# Autodesk Inventor assembly: case v3
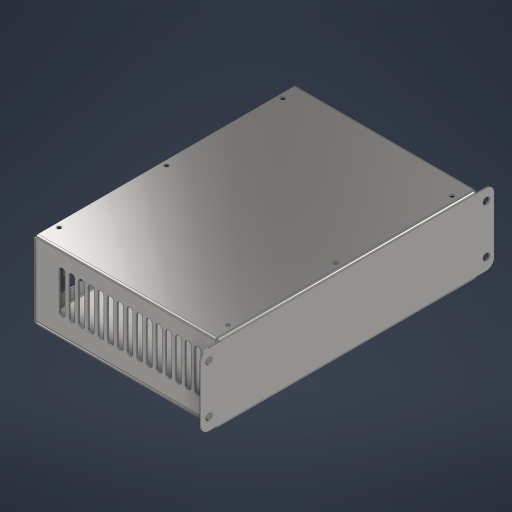
[picture p0: Inventor's stored thumbnail of the model, 512x512]
Saved by Autodesk Inventor 2024.2 (Build 282272000, 272)
## iProperties
Created: 2025-01-23
Part Number: case v3
Document SubType Name: Assembly
Designer: voids
Author: voids
## Documents named in this file (7)
- C:\Users\voids\Documents\GitHub\drive-hardware-dev\manufacturing\case v3.iam
- C:\Users\voids\Documents\GitHub\drive-hardware-dev\manufacturing\case v3 cover.ipt
- C:\Users\voids\Documents\GitHub\drive-hardware-dev\manufacturing\case v3.ipt
- C:\Users\voids\Documents\GitHub\drive-hardware-dev\manufacturing\simple step\HV servo drive v1r2\HV servo drive v1_PCB.ipt
- C:\Users\voids\Documents\GitHub\drive-hardware-dev\manufacturing\SanAce_9GA_40x20_RBD.ipt
- C:\Users\voids\Documents\GitHub\drive-hardware-dev\manufacturing\simple step\95185A110_Zinc-Plated Steel Press-Fit Nut for Sheet Metal\95185A110_Zinc-Plated Steel Press-Fit Nut for Sheet Metal.ipt
- C:\Users\voids\Documents\GitHub\drive-hardware-dev\manufacturing\simple step\95185A340_Zinc-Plated Steel Press-Fit Nut for Sheet Metal\95185A340_Zinc-Plated Steel Press-Fit Nut for Sheet Metal.ipt
## Components (16 placed, 6 different names)
1. case v3 cover:1 — Rigid:3, Rigid:10, Rigid:11, Rigid:12, Rigid:13
2. case v3:1 — Mate:1, Mate:2, Flush:1, Rigid:1, Rigid:2, Rigid:3, Rigid:4, Rigid:5, Rigid:6, Rigid:7, Rigid:8, Rigid:9, Rotational:1
3. HV servo drive v1_PCB:1 — Mate:1, Mate:2, Flush:1
4. SanAce_9GA_40x20_RBD:1 — Rigid:1
5. SanAce_9GA_40x20_RBD:2 — Rigid:2
6. 95185A110_Zinc-Plated Steel Press-Fit Nut for Sheet Metal:1 — Rigid:5
7. 95185A110_Zinc-Plated Steel Press-Fit Nut for Sheet Metal:2 — Rigid:7
8. 95185A110_Zinc-Plated Steel Press-Fit Nut for Sheet Metal:3 — Rigid:6
9. 95185A110_Zinc-Plated Steel Press-Fit Nut for Sheet Metal:4 — Rigid:8
10. 95185A110_Zinc-Plated Steel Press-Fit Nut for Sheet Metal:5 — Rigid:9
11. 95185A110_Zinc-Plated Steel Press-Fit Nut for Sheet Metal:6 — Rigid:10
12. 95185A110_Zinc-Plated Steel Press-Fit Nut for Sheet Metal:7 — Rigid:12
13. 95185A110_Zinc-Plated Steel Press-Fit Nut for Sheet Metal:8 — Rigid:13
14. 95185A110_Zinc-Plated Steel Press-Fit Nut for Sheet Metal:9 — Rigid:11
15. 95185A110_Zinc-Plated Steel Press-Fit Nut for Sheet Metal:10 — Rigid:4
16. 95185A340_Zinc-Plated Steel Press-Fit Nut for Sheet Metal:1 — Rotational:1
## Relationships (17: WeldJoint 13, Mate 2, Flush 1, RevoluteJoint 1)
- Mate:1 (7.9375 mm): case v3:1 ↔ HV servo drive v1_PCB:1
- Mate:2: case v3:1 ↔ HV servo drive v1_PCB:1
- Flush:1: case v3:1 ↔ HV servo drive v1_PCB:1
- Rigid:1 [WeldJoint]: case v3:1 ↔ SanAce_9GA_40x20_RBD:1
- Rigid:2 [WeldJoint]: case v3:1 ↔ SanAce_9GA_40x20_RBD:2
- Rigid:3 [WeldJoint]: case v3 cover:1 ↔ case v3:1
- Rigid:4 [WeldJoint]: case v3:1 ↔ 95185A110_Zinc-Plated Steel Press-Fit Nut for Sheet Metal:10
- Rigid:5 [WeldJoint]: case v3:1 ↔ 95185A110_Zinc-Plated Steel Press-Fit Nut for Sheet Metal:1
- Rigid:6 [WeldJoint]: case v3:1 ↔ 95185A110_Zinc-Plated Steel Press-Fit Nut for Sheet Metal:3
- Rigid:7 [WeldJoint]: case v3:1 ↔ 95185A110_Zinc-Plated Steel Press-Fit Nut for Sheet Metal:2
- Rigid:8 [WeldJoint]: case v3:1 ↔ 95185A110_Zinc-Plated Steel Press-Fit Nut for Sheet Metal:4
- Rigid:9 [WeldJoint]: case v3:1 ↔ 95185A110_Zinc-Plated Steel Press-Fit Nut for Sheet Metal:5
- Rigid:10 [WeldJoint]: case v3 cover:1 ↔ 95185A110_Zinc-Plated Steel Press-Fit Nut for Sheet Metal:6
- Rigid:11 [WeldJoint]: case v3 cover:1 ↔ 95185A110_Zinc-Plated Steel Press-Fit Nut for Sheet Metal:9
- Rigid:12 [WeldJoint]: case v3 cover:1 ↔ 95185A110_Zinc-Plated Steel Press-Fit Nut for Sheet Metal:7
- Rigid:13 [WeldJoint]: case v3 cover:1 ↔ 95185A110_Zinc-Plated Steel Press-Fit Nut for Sheet Metal:8
- Rotational:1 [RevoluteJoint]: case v3:1 ↔ 95185A340_Zinc-Plated Steel Press-Fit Nut for Sheet Metal:1
